# Autodesk Inventor assembly: POM_T5_06
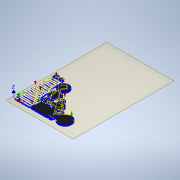
[picture p0: Inventor's stored thumbnail of the model, 180x180]
Saved by Autodesk Inventor 2020 (Build 240168000, 168)
## iProperties
Created: 2021-08-27
Part Number: POM_T5_06
Document SubType Name: Assembly
Designer: Masato
Author: Masato
## Documents named in this file (22)
- C:\Users\L20C1118 森　圭汰\Documents\220419_open\SUSTAINA-OP\Cam\POM_T5_06.iam
- C:\Users\L20C1118 森　圭汰\Documents\220419_open\SUSTAINA-OP\Cam\DisposableBoard.ipt
- C:\Users\L20C1118 森　圭汰\Documents\220419_open\SUSTAINA-OP\Jig\BackLink_diagonal_Jig.ipt
- C:\Users\L20C1118 森　圭汰\Documents\220419_open\SUSTAINA-OP\Jig\Foot_root_block_Jig.ipt
- C:\Users\L20C1118 森　圭汰\Documents\220419_open\SUSTAINA-OP\Jig\FrontLink_diagonal_Jig.ipt
- C:\Users\L20C1118 森　圭汰\Documents\220419_open\SUSTAINA-OP\Jig\Head_horn_frame_Jig.ipt
- C:\Users\L20C1118 森　圭汰\Documents\220419_open\SUSTAINA-OP\Jig\Leg_joint_yaw_frame_Jig.ipt
- C:\Users\L20C1118 森　圭汰\Documents\220419_open\SUSTAINA-OP\Jig\Shoulder_horn_frame_Jig.ipt
- C:\Users\L20C1118 森　圭汰\Documents\220419_open\SUSTAINA-OP\Jig\Trunk_chest_frame_Jig_1.ipt
- C:\Users\L20C1118 森　圭汰\Documents\220419_open\SUSTAINA-OP\Jig\Trunk_lower_side_frame_Jig.ipt
- C:\Users\L20C1118 森　圭汰\Documents\220419_open\SUSTAINA-OP\Jig\UpperArm_diagonal_Jig.ipt
- C:\Users\L20C1118 森　圭汰\Documents\220419_open\SUSTAINA-OP\SandBlastingJig\Foot_front_frame_SandBlastingJig_back.ipt
- C:\Users\L20C1118 森　圭汰\Documents\220419_open\SUSTAINA-OP\SandBlastingJig\Foot_front_frame_SandBlastingJig_front.ipt
- C:\Users\L20C1118 森　圭汰\Documents\220419_open\SUSTAINA-OP\SandBlastingJig\Leg_joint_slider_frame_SandBlastingJig_axis_back.ipt
- C:\Users\L20C1118 森　圭汰\Documents\220419_open\SUSTAINA-OP\SandBlastingJig\Leg_joint_slider_frame_SandBlastingJig_axis_front.ipt
- C:\Users\L20C1118 森　圭汰\Documents\220419_open\SUSTAINA-OP\SandBlastingJig\Leg_joint_slider_frame_SandBlastingJig_slider_back.ipt
- C:\Users\L20C1118 森　圭汰\Documents\220419_open\SUSTAINA-OP\SandBlastingJig\Leg_joint_slider_frame_SandBlastingJig_slider_front.ipt
- C:\Users\L20C1118 森　圭汰\Documents\220419_open\SUSTAINA-OP\SandBlastingJig\Leg_joint_yaw_frame_SandBlastingJig.ipt
- C:\Users\L20C1118 森　圭汰\Documents\220419_open\SUSTAINA-OP\SandBlastingJig\Outer_support_stand_SandBlastingJig.ipt
- C:\Users\L20C1118 森　圭汰\Documents\220419_open\SUSTAINA-OP\SandBlastingJig\Shoulder_horn_frame_SandBlastingJig.ipt
- C:\Users\L20C1118 森　圭汰\Documents\220419_open\SUSTAINA-OP\SandBlastingJig\Trunk_neck_frame_AND_Trunk_shoulder_frame_SandBlastingJig.ipt
- C:\Users\L20C1118 森　圭汰\Documents\220419_open\SUSTAINA-OP\SandBlastingJig\Trunk_servo_bottom_frame_SandBlastingJig.ipt
## Components (21 placed, 21 different names)
1. DisposableBoard:1 — メイト:2, メイト:1, フラッシュ:1, フラッシュ:2, メイト:4, メイト:5, メイト:6, メイト:7, メイト:8, メイト:9, メイト:10, メイト:11, メイト:12, メイト:13, メイト:14, メイト:15, メイト:16, メイト:17, メイト:18, メイト:19, メイト:20, メイト:21, メイト:22, メイト:23, フラッシュ:3, フラッシュ:4, 角度:1, 角度:2, 角度:3, 角度:4, 角度:5, 角度:6, 角度:7
2. BackLink_diagonal_Jig:1 — メイト:9, フラッシュ:10, メイト:29, フラッシュ:11, メイト:30
3. Foot_root_block_Jig:1 — メイト:12, フラッシュ:12, メイト:31, 正接:16, 正接:17, 正接:18
4. FrontLink_diagonal_Jig:1 — メイト:11, フラッシュ:5, メイト:24, フラッシュ:6, メイト:25, メイト:32
5. Head_horn_frame_Jig:1 — メイト:5, フラッシュ:8, フラッシュ:9, メイト:27, メイト:28
6. Leg_joint_yaw_frame_Jig:1 — メイト:10, フラッシュ:11, メイト:30, フラッシュ:12, メイト:31, 正接:8
7. Shoulder_horn_frame_Jig:1 — メイト:4, フラッシュ:9, メイト:28, フラッシュ:10, メイト:29, 正接:6
8. Trunk_chest_frame_Jig_1:1 — メイト:8, フラッシュ:6, メイト:25, フラッシュ:7, メイト:26, 正接:7
9. Trunk_lower_side_frame_Jig:1 — メイト:7, フラッシュ:3, フラッシュ:4, フラッシュ:5, メイト:24, フラッシュ:13
10. UpperArm_diagonal_Jig:1 — メイト:6, フラッシュ:7, メイト:26, フラッシュ:8, メイト:27
11. Foot_front_frame_SandBlastingJig_back:1 — メイト:22, 角度:4, 正接:12, 正接:13
12. Foot_front_frame_SandBlastingJig_front:1 — メイト:23, 角度:5, 正接:14, 正接:15
13. Leg_joint_slider_frame_SandBlastingJig_axis_back:1 — メイト:18, 角度:7, 正接:18, 正接:19
14. Leg_joint_slider_frame_SandBlastingJig_axis_front:1 — メイト:15, 角度:6, 正接:16, 正接:17, 正接:19
15. Leg_joint_slider_frame_SandBlastingJig_slider_back:1 — メイト:17, メイト:34, 正接:2, 正接:4, 正接:14
16. Leg_joint_slider_frame_SandBlastingJig_slider_front:1 — メイト:19, メイト:33, 正接:5, 正接:7, 正接:11
17. Leg_joint_yaw_frame_SandBlastingJig:1 — メイト:20, 正接:10, 正接:11, 正接:13
18. Outer_support_stand_SandBlastingJig:1 — メイト:16, 角度:1, 正接:3, 正接:4
19. Shoulder_horn_frame_SandBlastingJig:1 — メイト:21, 角度:3, 正接:8, 正接:9
20. Trunk_neck_frame_AND_Trunk_shoulder_frame_SandBlastingJig:1 — メイト:14, 正接:5, 角度:2, 正接:6, 正接:9, 正接:12
21. Trunk_servo_bottom_frame_SandBlastingJig:1 — メイト:13, フラッシュ:13, メイト:32, メイト:33, メイト:34, 正接:2, 正接:3, 正接:10, 正接:15
## Relationships (71: Mate 33, Tangent 18, Flush 13, Angle 7)
- メイト:2 [Mate]: DisposableBoard:1
- メイト:1 [Mate]: DisposableBoard:1
- フラッシュ:1 [Flush]: DisposableBoard:1
- フラッシュ:2 [Flush]: DisposableBoard:1
- メイト:4 [Mate]: DisposableBoard:1 ↔ Shoulder_horn_frame_Jig:1
- メイト:5 [Mate]: DisposableBoard:1 ↔ Head_horn_frame_Jig:1
- メイト:6 [Mate]: DisposableBoard:1 ↔ UpperArm_diagonal_Jig:1
- メイト:7 [Mate]: DisposableBoard:1 ↔ Trunk_lower_side_frame_Jig:1
- メイト:8 [Mate]: DisposableBoard:1 ↔ Trunk_chest_frame_Jig_1:1
- メイト:9 [Mate]: DisposableBoard:1 ↔ BackLink_diagonal_Jig:1
- メイト:10 [Mate]: DisposableBoard:1 ↔ Leg_joint_yaw_frame_Jig:1
- メイト:11 [Mate]: DisposableBoard:1 ↔ FrontLink_diagonal_Jig:1
- メイト:12 [Mate]: DisposableBoard:1 ↔ Foot_root_block_Jig:1
- メイト:13 [Mate]: DisposableBoard:1 ↔ Trunk_servo_bottom_frame_SandBlastingJig:1
- メイト:14 [Mate]: DisposableBoard:1 ↔ Trunk_neck_frame_AND_Trunk_shoulder_frame_SandBlastingJig:1
- メイト:15 [Mate]: DisposableBoard:1 ↔ Leg_joint_slider_frame_SandBlastingJig_axis_front:1
- メイト:16 [Mate]: DisposableBoard:1 ↔ Outer_support_stand_SandBlastingJig:1
- メイト:17 [Mate]: DisposableBoard:1 ↔ Leg_joint_slider_frame_SandBlastingJig_slider_back:1
- メイト:18 [Mate]: DisposableBoard:1 ↔ Leg_joint_slider_frame_SandBlastingJig_axis_back:1
- メイト:19 [Mate]: DisposableBoard:1 ↔ Leg_joint_slider_frame_SandBlastingJig_slider_front:1
- メイト:20 [Mate]: DisposableBoard:1 ↔ Leg_joint_yaw_frame_SandBlastingJig:1
- メイト:21 [Mate]: DisposableBoard:1 ↔ Shoulder_horn_frame_SandBlastingJig:1
- メイト:22 [Mate]: DisposableBoard:1 ↔ Foot_front_frame_SandBlastingJig_back:1
- メイト:23 [Mate]: DisposableBoard:1 ↔ Foot_front_frame_SandBlastingJig_front:1
- フラッシュ:3 [Flush] (2.5 mm): DisposableBoard:1 ↔ Trunk_lower_side_frame_Jig:1
- フラッシュ:4 [Flush] (-2.5 mm): DisposableBoard:1 ↔ Trunk_lower_side_frame_Jig:1
- フラッシュ:5 [Flush]: FrontLink_diagonal_Jig:1 ↔ Trunk_lower_side_frame_Jig:1
- メイト:24 [Mate] (2.5 mm): FrontLink_diagonal_Jig:1 ↔ Trunk_lower_side_frame_Jig:1
- フラッシュ:6 [Flush]: FrontLink_diagonal_Jig:1 ↔ Trunk_chest_frame_Jig_1:1
- メイト:25 [Mate] (2.5 mm): FrontLink_diagonal_Jig:1 ↔ Trunk_chest_frame_Jig_1:1
- フラッシュ:7 [Flush]: Trunk_chest_frame_Jig_1:1 ↔ UpperArm_diagonal_Jig:1
- メイト:26 [Mate] (2.5 mm): Trunk_chest_frame_Jig_1:1 ↔ UpperArm_diagonal_Jig:1
- フラッシュ:8 [Flush]: Head_horn_frame_Jig:1 ↔ UpperArm_diagonal_Jig:1
- フラッシュ:9 [Flush]: Head_horn_frame_Jig:1 ↔ Shoulder_horn_frame_Jig:1
- メイト:27 [Mate] (2.5 mm): Head_horn_frame_Jig:1 ↔ UpperArm_diagonal_Jig:1
- メイト:28 [Mate] (2.5 mm): Head_horn_frame_Jig:1 ↔ Shoulder_horn_frame_Jig:1
- フラッシュ:10 [Flush]: BackLink_diagonal_Jig:1 ↔ Shoulder_horn_frame_Jig:1
- メイト:29 [Mate] (2.5 mm): BackLink_diagonal_Jig:1 ↔ Shoulder_horn_frame_Jig:1
- フラッシュ:11 [Flush]: BackLink_diagonal_Jig:1 ↔ Leg_joint_yaw_frame_Jig:1
- メイト:30 [Mate] (2.5 mm): BackLink_diagonal_Jig:1 ↔ Leg_joint_yaw_frame_Jig:1
- フラッシュ:12 [Flush]: Foot_root_block_Jig:1 ↔ Leg_joint_yaw_frame_Jig:1
- メイト:31 [Mate] (2.5 mm): Foot_root_block_Jig:1 ↔ Leg_joint_yaw_frame_Jig:1
- フラッシュ:13 [Flush]: Trunk_lower_side_frame_Jig:1 ↔ Trunk_servo_bottom_frame_SandBlastingJig:1
- メイト:32 [Mate] (2.5 mm): FrontLink_diagonal_Jig:1 ↔ Trunk_servo_bottom_frame_SandBlastingJig:1
- メイト:33 [Mate] (2.5 mm): Leg_joint_slider_frame_SandBlastingJig_slider_front:1 ↔ Trunk_servo_bottom_frame_SandBlastingJig:1
- メイト:34 [Mate] (2.5 mm): Leg_joint_slider_frame_SandBlastingJig_slider_back:1 ↔ Trunk_servo_bottom_frame_SandBlastingJig:1
- 正接:2 [Tangent]: Leg_joint_slider_frame_SandBlastingJig_slider_back:1 ↔ Trunk_servo_bottom_frame_SandBlastingJig:1
- 角度:1 [Angle] (0 deg): DisposableBoard:1 ↔ Outer_support_stand_SandBlastingJig:1
- 正接:3 [Tangent]: Outer_support_stand_SandBlastingJig:1 ↔ Trunk_servo_bottom_frame_SandBlastingJig:1
- 正接:4 [Tangent] (2.5 mm): Leg_joint_slider_frame_SandBlastingJig_slider_back:1 ↔ Outer_support_stand_SandBlastingJig:1
- 正接:5 [Tangent] (2.5 mm): Leg_joint_slider_frame_SandBlastingJig_slider_front:1 ↔ Trunk_neck_frame_AND_Trunk_shoulder_frame_SandBlastingJig:1
- 角度:2 [Angle] (0 deg): DisposableBoard:1 ↔ Trunk_neck_frame_AND_Trunk_shoulder_frame_SandBlastingJig:1
- 正接:6 [Tangent] (2.5 mm): Shoulder_horn_frame_Jig:1 ↔ Trunk_neck_frame_AND_Trunk_shoulder_frame_SandBlastingJig:1
- 正接:7 [Tangent] (2.5 mm): Trunk_chest_frame_Jig_1:1 ↔ Leg_joint_slider_frame_SandBlastingJig_slider_front:1
- 角度:3 [Angle] (0 deg): DisposableBoard:1 ↔ Shoulder_horn_frame_SandBlastingJig:1
- 正接:8 [Tangent] (2.5 mm): Leg_joint_yaw_frame_Jig:1 ↔ Shoulder_horn_frame_SandBlastingJig:1
- 正接:9 [Tangent] (2.5 mm): Shoulder_horn_frame_SandBlastingJig:1 ↔ Trunk_neck_frame_AND_Trunk_shoulder_frame_SandBlastingJig:1
- 正接:10 [Tangent] (2.5 mm): Leg_joint_yaw_frame_SandBlastingJig:1 ↔ Trunk_servo_bottom_frame_SandBlastingJig:1
- 正接:11 [Tangent] (2.5 mm): Leg_joint_slider_frame_SandBlastingJig_slider_front:1 ↔ Leg_joint_yaw_frame_SandBlastingJig:1
- 角度:4 [Angle] (0 deg): DisposableBoard:1 ↔ Foot_front_frame_SandBlastingJig_back:1
- 正接:12 [Tangent] (2.5 mm): Foot_front_frame_SandBlastingJig_back:1 ↔ Trunk_neck_frame_AND_Trunk_shoulder_frame_SandBlastingJig:1
- 正接:13 [Tangent] (2.5 mm): Foot_front_frame_SandBlastingJig_back:1 ↔ Leg_joint_yaw_frame_SandBlastingJig:1
- 角度:5 [Angle] (0 deg): DisposableBoard:1 ↔ Foot_front_frame_SandBlastingJig_front:1
- 正接:14 [Tangent] (2.5 mm): Foot_front_frame_SandBlastingJig_front:1 ↔ Leg_joint_slider_frame_SandBlastingJig_slider_back:1
- 正接:15 [Tangent] (2.5 mm): Foot_front_frame_SandBlastingJig_front:1 ↔ Trunk_servo_bottom_frame_SandBlastingJig:1
- 角度:6 [Angle] (0 deg): DisposableBoard:1 ↔ Leg_joint_slider_frame_SandBlastingJig_axis_front:1
- 正接:16 [Tangent] (2.5 mm): Foot_root_block_Jig:1 ↔ Leg_joint_slider_frame_SandBlastingJig_axis_front:1
- 正接:17 [Tangent]: Foot_root_block_Jig:1 ↔ Leg_joint_slider_frame_SandBlastingJig_axis_front:1
- 角度:7 [Angle] (0 deg): DisposableBoard:1 ↔ Leg_joint_slider_frame_SandBlastingJig_axis_back:1
- 正接:18 [Tangent] (2.5 mm): Foot_root_block_Jig:1 ↔ Leg_joint_slider_frame_SandBlastingJig_axis_back:1
- 正接:19 [Tangent] (2.5 mm): Leg_joint_slider_frame_SandBlastingJig_axis_back:1 ↔ Leg_joint_slider_frame_SandBlastingJig_axis_front:1
